# Autodesk Inventor assembly: PIP-Boy 6400 Mk_I Full Assembly
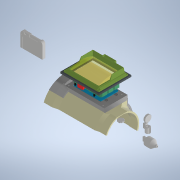
[picture p0: Inventor's stored thumbnail of the model, 180x180]
Saved by Autodesk Inventor 2021 (Build 250183000, 183)
## iProperties
Created: 2021-04-29
Part Number: PIP-Boy 6400 Mk_I Full Assembly
Document SubType Name: Assembly
Designer: trent
Author: trent
## Documents named in this file (13)
- C:\Users\EmeraldLeeTiger\OneDrive - wmpenn.edu\Personal\PIP-Boy 6400 Mk.I\PIP-Boy 6400 Mk_I Full Assembly.iam
- C:\Users\EmeraldLeeTiger\OneDrive - wmpenn.edu\Personal\PIP-Boy 6400 Mk.I\PIP-Boy 6400 Mk_I Computer Subassembly.iam
- C:\Users\EmeraldLeeTiger\OneDrive - wmpenn.edu\Personal\PIP-Boy 6400 Mk.I\ArmPiece_TopHalf.ipt
- C:\Users\EmeraldLeeTiger\OneDrive - wmpenn.edu\Personal\PIP-Boy 6400 Mk.I\MainHousing_BackMainShell.ipt
- C:\Users\EmeraldLeeTiger\OneDrive - wmpenn.edu\Personal\PIP-Boy 6400 Mk.I\MainHousing_FrontMainShell.ipt
- C:\Users\EmeraldLeeTiger\OneDrive - wmpenn.edu\Personal\PIP-Boy 6400 Mk.I\MainHousing_Screen Acrylic.ipt
- C:\Users\EmeraldLeeTiger\OneDrive - wmpenn.edu\Personal\PIP-Boy 6400 Mk.I\MainHousing_Screen Visor.ipt
- C:\Users\EmeraldLeeTiger\OneDrive - wmpenn.edu\Personal\PIP-Boy 6400 Mk.I\Dial_Main-Sub Menu Dial.ipt
- C:\Users\EmeraldLeeTiger\OneDrive - wmpenn.edu\Personal\PIP-Boy 6400 Mk.I\Button_SelectButton.ipt
- C:\Users\EmeraldLeeTiger\OneDrive - wmpenn.edu\Personal\PIP-Boy 6400 Mk.I\Dial_Radio.ipt
- C:\Users\EmeraldLeeTiger\OneDrive - wmpenn.edu\Personal\PIP-Boy 6400 Mk.I\Dial_InventoryScroll.ipt
- C:\Users\EmeraldLeeTiger\OneDrive - wmpenn.edu\Personal\PIP-Boy 6400 Mk.I\MainHousing_DataPlug.ipt
- C:\Users\EmeraldLeeTiger\OneDrive - wmpenn.edu\Personal\PIP-Boy 6400 Mk.I\Holotape.iam
## Components (12 placed, 12 different names)
1. PIP-Boy 6400 Mk_I Computer Subassembly:1 [sub-assembly] — Mate:1, Mate:2, Mate:3, Mate:13, Mate:14, Mate:15
2. ArmPiece_TopHalf:1 — Mate:4, Mate:5, Mate:6
3. MainHousing_BackMainShell:1 — Mate:1, Mate:2, Mate:3, Mate:4, Mate:5, Mate:6
4. MainHousing_FrontMainShell:1 — Mate:10, Mate:11, Mate:12, Mate:13, Mate:14
5. MainHousing_Screen Acrylic:1 — Mate:7, Mate:8, Mate:9, Mate:15
6. MainHousing_Screen Visor:1 — Mate:7, Mate:8, Mate:9, Mate:10, Mate:11, Mate:12
7. Dial_Main-Sub Menu Dial:1
8. Button_SelectButton:1
9. Dial_Radio:1
10. Dial_InventoryScroll:1
11. MainHousing_DataPlug:1
12. Holotape:1 [sub-assembly]
## Relationships (15: Mate 15)
- Mate:1: PIP-Boy 6400 Mk_I Computer Subassembly:1 ↔ MainHousing_BackMainShell:1
- Mate:2: PIP-Boy 6400 Mk_I Computer Subassembly:1 ↔ MainHousing_BackMainShell:1
- Mate:3: PIP-Boy 6400 Mk_I Computer Subassembly:1 ↔ MainHousing_BackMainShell:1
- Mate:4: ArmPiece_TopHalf:1 ↔ MainHousing_BackMainShell:1
- Mate:5: ArmPiece_TopHalf:1 ↔ MainHousing_BackMainShell:1
- Mate:6: ArmPiece_TopHalf:1 ↔ MainHousing_BackMainShell:1
- Mate:7: MainHousing_Screen Acrylic:1 ↔ MainHousing_Screen Visor:1
- Mate:8: MainHousing_Screen Acrylic:1 ↔ MainHousing_Screen Visor:1
- Mate:9: MainHousing_Screen Acrylic:1 ↔ MainHousing_Screen Visor:1
- Mate:10: MainHousing_FrontMainShell:1 ↔ MainHousing_Screen Visor:1
- Mate:11: MainHousing_FrontMainShell:1 ↔ MainHousing_Screen Visor:1
- Mate:12: MainHousing_FrontMainShell:1 ↔ MainHousing_Screen Visor:1
- Mate:13 (7 mm): PIP-Boy 6400 Mk_I Computer Subassembly:1 ↔ MainHousing_FrontMainShell:1
- Mate:14 (1.125 mm): PIP-Boy 6400 Mk_I Computer Subassembly:1 ↔ MainHousing_FrontMainShell:1
- Mate:15 (2 mm): PIP-Boy 6400 Mk_I Computer Subassembly:1 ↔ MainHousing_Screen Acrylic:1
